# Autodesk Inventor assembly: Pancake_Pneumatic_Cylinder_217-2778 (3)
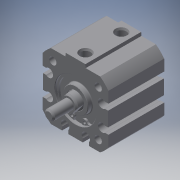
[picture p0: Inventor's stored thumbnail of the model, 180x180]
Saved by Autodesk Inventor 2019.4 (Build 234330000, 330)
## iProperties
Created: 2014-08-06
Part Number: Pancake_Pneumatic_Cylinder_217-2778 (3)
Description: STEP AP203
Document SubType Name: Assembly
Designer: mavericks
Title: 217-2778-001 Rev2.STEP
Revision Number: ANY
Sending System: SolidWorks 2014
Preprocessor: SwSTEP 2.0
## Documents named in this file (4)
- T:\EIT\2020 Infinite Recharge\2020 ROBOT\COMMON PARTS\AIR CYLINDERS\Pancake_Pneumatic_Cylinder_217-2778 (3).iam
- T:\EIT\2020 Infinite Recharge\2020 ROBOT\COMMON PARTS\AIR CYLINDERS\217-2778-NCQ8A075-050M_NCQ8 Tube_075A.ipt
- T:\EIT\2020 Infinite Recharge\2020 ROBOT\COMMON PARTS\AIR CYLINDERS\217-2778-NCQ8A075-050M_NCQ8 Rod_075M.ipt
- T:\EIT\2020 Infinite Recharge\2020 ROBOT\COMMON PARTS\AIR CYLINDERS\217-2778-NCQ8A075-050M_Snap Ring_075.ipt
## Components (3 placed, 3 different names)
1. 217-2778-NCQ8A075-050M_NCQ8 Tube_075A_1 — Insert:1
2. 217-2778-NCQ8A075-050M_NCQ8 Rod_075M_2 — Insert:1
3. 217-2778-NCQ8A075-050M_Snap Ring_075_3
## Relationships (1: Insert 1)
- Insert:1: 217-2778-NCQ8A075-050M_NCQ8 Tube_075A_1 ↔ 217-2778-NCQ8A075-050M_NCQ8 Rod_075M_2
